# Autodesk Inventor assembly: am-2256 4 in HiGrip Wheel
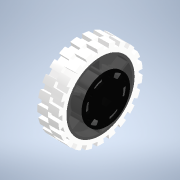
[picture p0: Inventor's stored thumbnail of the model, 180x180]
Saved by Autodesk Inventor 2020 (Build 240168000, 168)
## iProperties
Created: 2012-12-03
Part Number: am-2256 4 in HiGrip Wheel
Description: STEP AP214
Document SubType Name: Assembly
Designer: autum
Sending System: SolidWorks 2010
Preprocessor: SwSTEP 2.0
Title: 4 in HiGrip Wheel.STEP
Revision Number: ANY
## Documents named in this file (4)
- C:\Users\autum\Google Drive\Iron Riders 4180 (Roosevelt Robotics)\2019-2020\Build_Design\Robot 2020 (1)\Manipulators\Hooded Shooter (Protected Zone)\am-2256 4 in HiGrip Wheel.iam
- C:\Users\autum\Google Drive\Iron Riders 4180 (Roosevelt Robotics)\2019-2020\Build_Design\Robot 2020 (1)\Manipulators\Hooded Shooter (Protected Zone)\4in 2013 Hub.ipt
- C:\Users\autum\Google Drive\Iron Riders 4180 (Roosevelt Robotics)\2019-2020\Build_Design\Robot 2020 (1)\Manipulators\Hooded Shooter (Protected Zone)\4 in tread.ipt
- C:\Users\autum\Google Drive\Iron Riders 4180 (Roosevelt Robotics)\2019-2020\Build_Design\Robot 2020 (1)\Manipulators\Hooded Shooter (Protected Zone)\1_2_Hex_Bore_Aluminum_VersaHub_217-2592.ipt
## Components (4 placed, 3 different names)
1. 4in 2013 Hub_1 — Insert:1, Insert:2
2. 4 in tread_2
3. 1_2_Hex_Bore_Aluminum_VersaHub_217-2592:1 — Insert:1
4. 1_2_Hex_Bore_Aluminum_VersaHub_217-2592:2 — Insert:2
## Relationships (2: Insert 2)
- Insert:1: 4in 2013 Hub_1 ↔ 1_2_Hex_Bore_Aluminum_VersaHub_217-2592:1
- Insert:2: 4in 2013 Hub_1 ↔ 1_2_Hex_Bore_Aluminum_VersaHub_217-2592:2
